# Autodesk Inventor assembly: DriveUnit
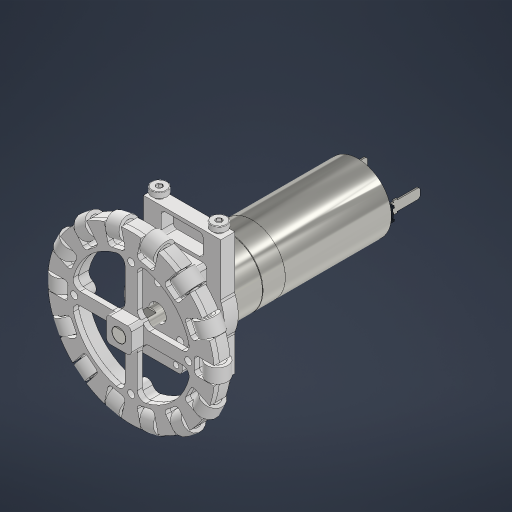
[picture p0: Inventor's stored thumbnail of the model, 512x512]
Saved by Autodesk Inventor 2024.2 (Build 282272000, 272)
## iProperties
Created: 2023-12-20
Part Number: DriveUnit
Document SubType Name: Assembly
Designer: Hanaoka
Author: Hanaoka
## Documents named in this file (7)
- G:\共有ドライブ\reRo\05_個人\hanaoka\inventor\DriveUnit\DriveUnit.iam
- G:\共有ドライブ\reRo\05_個人\hanaoka\inventor\DriveUnit\dcx19s_gpx19c\dcx19s_gpx19c.iam
- G:\共有ドライブ\reRo\05_個人\hanaoka\inventor\DriveUnit\OmniWheel.iam
- G:\共有ドライブ\reRo\05_個人\hanaoka\inventor\DriveUnit\MotorMount_sub.ipt
- G:\共有ドライブ\reRo\05_個人\hanaoka\inventor\DriveUnit\MotorMount_main.ipt
- G:\共有ドライブ\reRo\05_個人\hanaoka\inventor\Screw\M2.6x8\M2.6x8.ipt
- G:\共有ドライブ\reRo\05_個人\hanaoka\inventor\Screw\M2xL6\M2x6.ipt
## Components (12 placed, 6 different names)
1. dcx19s_gpx19c:1 [sub-assembly] — フラッシュ:1, フラッシュ:2, 正接:1, 回転:1, メイト:1, メイト:2, メイト:3
2. OmniWheel:1 [sub-assembly] — 回転:1
3. MotorMount_sub:1 — メイト:1, メイト:2, メイト:3, メイト:4, メイト:5, メイト:6
4. MotorMount_main:1 — メイト:4, メイト:5, メイト:6, 挿入:1, 挿入:2, 挿入:3, 挿入:4, 挿入:5, 挿入:6, 挿入:7, 挿入:8
5. M2.6x8:1 — 挿入:1
6. M2.6x8:2 — 挿入:4
7. M2.6x8:3 — 挿入:2
8. M2.6x8:4 — 挿入:3
9. M2x6:1 — 挿入:6
10. M2x6:2 — 挿入:7
11. M2x6:3 — 挿入:8
12. M2x6:4 — 挿入:5
## Relationships (18: Insert 8, Mate 6, Flush 2, Tangent 1, RevoluteJoint 1)
- フラッシュ:1 [Flush]: dcx19s_gpx19c:1
- フラッシュ:2 [Flush] (-1.5 mm): dcx19s_gpx19c:1
- 正接:1 [Tangent] (-2 mm): dcx19s_gpx19c:1
- 回転:1 [RevoluteJoint]: dcx19s_gpx19c:1 ↔ OmniWheel:1
- メイト:1 [Mate]: dcx19s_gpx19c:1 ↔ MotorMount_sub:1
- メイト:2 [Mate]: dcx19s_gpx19c:1 ↔ MotorMount_sub:1
- メイト:3 [Mate]: dcx19s_gpx19c:1 ↔ MotorMount_sub:1
- メイト:4 [Mate]: MotorMount_sub:1 ↔ MotorMount_main:1
- メイト:5 [Mate]: MotorMount_sub:1 ↔ MotorMount_main:1
- メイト:6 [Mate]: MotorMount_sub:1 ↔ MotorMount_main:1
- 挿入:1 [Insert] (1 mm): MotorMount_main:1 ↔ M2.6x8:1
- 挿入:2 [Insert] (1 mm): MotorMount_main:1 ↔ M2.6x8:3
- 挿入:3 [Insert] (1 mm): MotorMount_main:1 ↔ M2.6x8:4
- 挿入:4 [Insert] (1 mm): MotorMount_main:1 ↔ M2.6x8:2
- 挿入:5 [Insert]: MotorMount_main:1 ↔ M2x6:4
- 挿入:6 [Insert]: MotorMount_main:1 ↔ M2x6:1
- 挿入:7 [Insert]: MotorMount_main:1 ↔ M2x6:2
- 挿入:8 [Insert]: MotorMount_main:1 ↔ M2x6:3
